# Autodesk Inventor assembly: Garra_CH
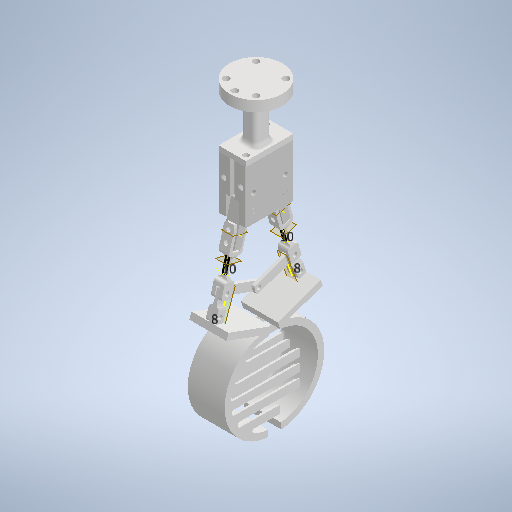
[picture p0: Inventor's stored thumbnail of the model, 512x512]
Saved by Autodesk Inventor 2025 (Build 290162000, 162)
## iProperties
Created: 2025-07-17
Part Number: Garra_CH
Document SubType Name: Assembly
Designer: acer
Author: acer
## Documents named in this file (7)
- E:\Documents\Universidad\10mo Semestre\Robotica\Garra_C\Garra_CH.iam
- E:\Documents\Universidad\10mo Semestre\Robotica\Garra_C\Acoplador (1).ipt
- E:\Documents\Universidad\10mo Semestre\Robotica\Garra_C\Acoplador.ipt
- E:\Documents\Universidad\10mo Semestre\Robotica\Garra_C\Flange.ipt
- E:\Documents\Universidad\10mo Semestre\Robotica\Garra_C\L_1 (1).ipt
- E:\Documents\Universidad\10mo Semestre\Robotica\Garra_C\MCHA-20.iam
- C:\Users\acer\OneDrive\Documentos\Pinza.ipt
## Components (8 placed, 6 different names)
1. Acoplador (1):1 — Rígido:3, Insertar:1, Ángulo:1
2. Acoplador:1 — Rígido:2, Insertar:2, Ángulo:2
3. Flange:1 — Rígido:1
4. L_1 (1):1 — Insertar:1, Ángulo:1, De rotación:1
5. MCHA-20:1 [sub-assembly] — Rígido:1, Rígido:2, Rígido:3
6. L_1 (1):2 — Insertar:2, Ángulo:2, De rotación:2
7. Pinza:1 — De rotación:1
8. Pinza:2 — De rotación:2
## Relationships (9: WeldJoint 3, Insert 2, Angle 2, RevoluteJoint 2)
- Rígido:1 [WeldJoint]: Flange:1 ↔ MCHA-20:1
- Rígido:2 [WeldJoint]: Acoplador:1 ↔ MCHA-20:1
- Rígido:3 [WeldJoint]: Acoplador (1):1 ↔ MCHA-20:1
- Insertar:1: Acoplador (1):1 ↔ L_1 (1):1
- Ángulo:1 [Angle] (-85 deg): Acoplador (1):1 ↔ L_1 (1):1
- Insertar:2: Acoplador:1 ↔ L_1 (1):2
- Ángulo:2 [Angle] (185 deg): Acoplador:1 ↔ L_1 (1):2
- De rotación:1 [RevoluteJoint]: L_1 (1):1 ↔ Pinza:1
- De rotación:2 [RevoluteJoint]: L_1 (1):2 ↔ Pinza:2
